# Autodesk Inventor assembly: 2020 Flex Seal Chasis
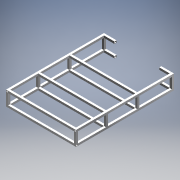
[picture p0: Inventor's stored thumbnail of the model, 180x180]
Saved by Autodesk Inventor 2019.4 (Build 234330000, 330)
## iProperties
Created: 2019-01-05
Part Number: 2020 Flex Seal Chasis
Document SubType Name: Assembly
Designer: Jacob's Laptop
Mass: 5184.97 g
Surface Area: 12177.4 cm^2
Volume: 1920.36 cm^3
Density: 2.7 g/cm^3
Author: Jacob's Laptop
## Documents named in this file (7)
- D:\FIRST FRC\Synthesis Robots\Epsilon\Chasis\2020 Flex Seal Chasis.iam
- D:\FIRST FRC\Synthesis Robots\Epsilon\Chasis\Chasis Long Length.ipt
- D:\FIRST FRC\Synthesis Robots\Epsilon\Chasis\Chasis Short Length.ipt
- D:\FIRST FRC\Synthesis Robots\Epsilon\Chasis\Chasis Hieght.ipt
- D:\FIRST FRC\Synthesis Robots\Epsilon\Chasis\Chasis Long Length 2.ipt
- D:\FIRST FRC\Synthesis Robots\Epsilon\Chasis\Chasis Short Length 2.ipt
- D:\FIRST FRC\Synthesis Robots\Epsilon\Chasis\Chasis Hieght 2.ipt
## Components (22 placed, 6 different names)
1. Chasis Short Length:1 — Mate:20, Flush:27, Flush:35
2. Chasis Hieght:1 — Mate:11, Flush:21, Flush:22, Mate:22, Flush:45
3. Chasis Hieght:4 — Mate:21, Flush:26, Flush:33, Flush:34, Mate:24, Flush:36
4. Chasis Long Length:3 — Mate:11, Flush:21, Flush:22, Flush:33, Flush:34, Mate:24, Mate:25, Flush:37, Mate:26, Flush:38
5. Chasis Hieght:5 — Flush:46, Mate:31, Flush:47, Flush:52, Flush:60
6. Chasis Hieght:7 — Flush:43, Flush:44, Mate:30, Flush:47, Flush:58
7. Chasis Long Length 2:1 — Mate:20, Mate:21, Flush:26, Flush:27, Flush:35, Mate:27, Flush:39, Flush:40, Mate:31, Mate:34, Flush:51, Flush:53, Mate:35, Mate:38, Flush:61, Flush:62
8. Chasis Long Length 2:3 — Mate:22, Mate:28, Flush:41, Flush:42, Flush:43, Flush:45, Mate:32, Flush:48, Mate:40, Flush:65, Flush:66
9. Chasis Short Length 2:1 — Mate:25, Flush:36, Flush:37, Mate:29, Flush:46, Mate:33, Flush:49, Flush:64
10. Chasis Short Length 2:2 — Mate:26, Flush:38, Flush:44, Mate:30, Mate:36, Flush:55, Mate:37, Flush:57, Flush:68
11. Chasis Hieght 2:1 — Mate:27, Flush:39, Flush:40, Mate:29, Mate:39, Flush:63
12. Chasis Hieght 2:2 — Mate:28, Flush:41, Flush:42, Mate:41, Flush:67
13. Chasis Hieght:8 — Mate:33, Flush:49, Flush:50, Flush:54, Flush:59
14. Chasis Hieght:9 — Mate:32, Flush:48, Flush:50, Flush:56
15. Chasis Short Length:2 — Flush:53, Mate:35, Flush:54
16. Chasis Short Length:3 — Mate:34, Flush:51, Flush:52
17. Chasis Short Length:4 — Mate:36, Flush:55, Flush:56, Flush:59
18. Chasis Short Length:5 — Mate:37, Flush:57, Flush:58, Flush:60
19. Chasis Hieght:10 — Mate:38, Flush:61, Flush:62
20. Chasis Hieght:11 — Mate:39, Flush:63, Flush:64
21. Chasis Hieght:12 — Mate:41, Flush:67, Flush:68
22. Chasis Hieght:13 — Mate:40, Flush:65, Flush:66
## Relationships (62: Flush 40, Mate 22)
- Mate:11: Chasis Hieght:1 ↔ Chasis Long Length:3
- Flush:21: Chasis Hieght:1 ↔ Chasis Long Length:3
- Flush:22: Chasis Hieght:1 ↔ Chasis Long Length:3
- Mate:20: Chasis Short Length:1 ↔ Chasis Long Length 2:1
- Mate:21: Chasis Hieght:4 ↔ Chasis Long Length 2:1
- Flush:26: Chasis Hieght:4 ↔ Chasis Long Length 2:1
- Flush:27: Chasis Short Length:1 ↔ Chasis Long Length 2:1
- Mate:22: Chasis Hieght:1 ↔ Chasis Long Length 2:3
- Flush:33: Chasis Hieght:4 ↔ Chasis Long Length:3
- Flush:34: Chasis Hieght:4 ↔ Chasis Long Length:3
- Flush:35: Chasis Short Length:1 ↔ Chasis Long Length 2:1
- Mate:24: Chasis Hieght:4 ↔ Chasis Long Length:3
- Mate:25: Chasis Long Length:3 ↔ Chasis Short Length 2:1
- Flush:36: Chasis Hieght:4 ↔ Chasis Short Length 2:1
- Flush:37: Chasis Long Length:3 ↔ Chasis Short Length 2:1
- Mate:26: Chasis Long Length:3 ↔ Chasis Short Length 2:2
- Flush:38: Chasis Long Length:3 ↔ Chasis Short Length 2:2
- Mate:27: Chasis Long Length 2:1 ↔ Chasis Hieght 2:1
- Flush:39: Chasis Long Length 2:1 ↔ Chasis Hieght 2:1
- Flush:40: Chasis Long Length 2:1 ↔ Chasis Hieght 2:1
- Mate:28: Chasis Long Length 2:3 ↔ Chasis Hieght 2:2
- Flush:41: Chasis Long Length 2:3 ↔ Chasis Hieght 2:2
- Flush:42: Chasis Long Length 2:3 ↔ Chasis Hieght 2:2
- Mate:29: Chasis Short Length 2:1 ↔ Chasis Hieght 2:1
- Flush:43: Chasis Hieght:7 ↔ Chasis Long Length 2:3
- Flush:44: Chasis Hieght:7 ↔ Chasis Short Length 2:2
- Flush:45: Chasis Hieght:1 ↔ Chasis Long Length 2:3
- Mate:30: Chasis Hieght:7 ↔ Chasis Short Length 2:2
- Flush:46: Chasis Hieght:5 ↔ Chasis Short Length 2:1
- Mate:31: Chasis Hieght:5 ↔ Chasis Long Length 2:1
- Flush:47: Chasis Hieght:5 ↔ Chasis Hieght:7
- Mate:32: Chasis Long Length 2:3 ↔ Chasis Hieght:9
- Flush:48: Chasis Long Length 2:3 ↔ Chasis Hieght:9
- Mate:33: Chasis Short Length 2:1 ↔ Chasis Hieght:8
- Flush:49: Chasis Short Length 2:1 ↔ Chasis Hieght:8
- Flush:50: Chasis Hieght:8 ↔ Chasis Hieght:9
- Mate:34: Chasis Long Length 2:1 ↔ Chasis Short Length:3
- Flush:51: Chasis Long Length 2:1 ↔ Chasis Short Length:3
- Flush:52: Chasis Hieght:5 ↔ Chasis Short Length:3
- Flush:53: Chasis Long Length 2:1 ↔ Chasis Short Length:2
- Mate:35: Chasis Long Length 2:1 ↔ Chasis Short Length:2
- Flush:54: Chasis Hieght:8 ↔ Chasis Short Length:2
- Mate:36: Chasis Short Length 2:2 ↔ Chasis Short Length:4
- Flush:55: Chasis Short Length 2:2 ↔ Chasis Short Length:4
- Flush:56: Chasis Hieght:9 ↔ Chasis Short Length:4
- Mate:37: Chasis Short Length 2:2 ↔ Chasis Short Length:5
- Flush:57: Chasis Short Length 2:2 ↔ Chasis Short Length:5
- Flush:58: Chasis Hieght:7 ↔ Chasis Short Length:5
- Flush:59: Chasis Hieght:8 ↔ Chasis Short Length:4
- Flush:60: Chasis Hieght:5 ↔ Chasis Short Length:5
- Mate:38: Chasis Long Length 2:1 ↔ Chasis Hieght:10
- Flush:61: Chasis Long Length 2:1 ↔ Chasis Hieght:10
- Flush:62: Chasis Long Length 2:1 ↔ Chasis Hieght:10
- Mate:39: Chasis Hieght 2:1 ↔ Chasis Hieght:11
- Flush:63: Chasis Hieght 2:1 ↔ Chasis Hieght:11
- Flush:64: Chasis Short Length 2:1 ↔ Chasis Hieght:11
- Mate:40: Chasis Long Length 2:3 ↔ Chasis Hieght:13
- Flush:65: Chasis Long Length 2:3 ↔ Chasis Hieght:13
- Flush:66: Chasis Long Length 2:3 ↔ Chasis Hieght:13
- Mate:41: Chasis Hieght 2:2 ↔ Chasis Hieght:12
- Flush:67: Chasis Hieght 2:2 ↔ Chasis Hieght:12
- Flush:68: Chasis Short Length 2:2 ↔ Chasis Hieght:12
